# Autodesk Inventor assembly: mg996r_bottom
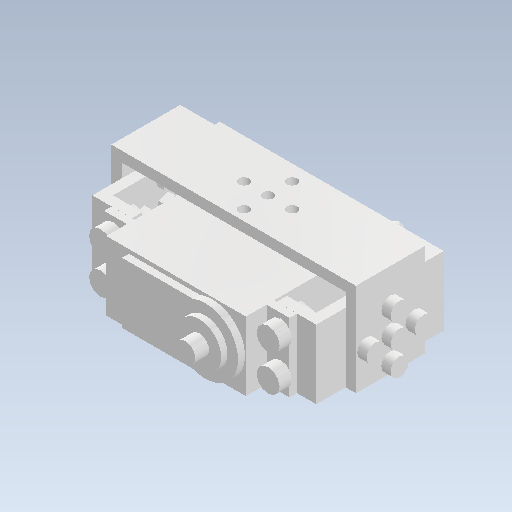
[picture p0: Inventor's stored thumbnail of the model, 512x512]
Saved by Autodesk Inventor 2021.4 (Build 254397000, 397)
## iProperties
Created: 2022-07-25
Part Number: mg996r_bottom
Document SubType Name: Assembly
Designer: isamu
Author: isamu
## Documents named in this file (5)
- D:\personal_projects\robot\inventor\2021_matlab_compat\mg996r_bottom.iam
- D:\personal_projects\robot\inventor\2021_matlab_compat\mg996r_servo_frame_with_axis.iam
- D:\personal_projects\robot\exports\frames\servo frame part 3.ipt
- D:\personal_projects\robot\exports\screws\m3x8.ipt
- D:\personal_projects\robot\exports\screws\m3 nuts.ipt
## Components (22 placed, 4 different names)
1. mg996r_servo_frame_with_axis:1 [sub-assembly] — Mate:1, Mate:2, Mate:3, Insert:11, Insert:12, Insert:13, Insert:14, Insert:15, Insert:16, Insert:17, Insert:18, Insert:19, Insert:20
2. servo frame part 3:1 — Mate:1, Mate:2, Mate:3, Insert:1, Insert:2, Insert:3, Insert:4, Insert:5, Insert:6, Insert:7, Insert:8, Insert:9, Insert:10
3. m3x8:1 — Insert:7
4. m3x8:2 — Insert:8
5. m3x8:3 — Insert:10
6. m3x8:4 — Insert:9
7. m3x8:5 — Insert:6
8. m3x8:6 — Insert:2
9. m3x8:7 — Insert:3
10. m3x8:8 — Insert:5
11. m3x8:9 — Insert:4
12. m3x8:10 — Insert:1
13. m3 nuts:1 — Insert:17
14. m3 nuts:2 — Insert:20
15. m3 nuts:3 — Insert:19
16. m3 nuts:4 — Insert:16
17. m3 nuts:5 — Insert:18
18. m3 nuts:6 — Insert:11
19. m3 nuts:7 — Insert:14
20. m3 nuts:8 — Insert:13
21. m3 nuts:9 — Insert:15
22. m3 nuts:10 — Insert:12
## Relationships (23: Insert 20, Mate 3)
- Mate:1: mg996r_servo_frame_with_axis:1 ↔ servo frame part 3:1
- Mate:2: mg996r_servo_frame_with_axis:1 ↔ servo frame part 3:1
- Mate:3: mg996r_servo_frame_with_axis:1 ↔ servo frame part 3:1
- Insert:1: servo frame part 3:1 ↔ m3x8:10
- Insert:2: servo frame part 3:1 ↔ m3x8:6
- Insert:3: servo frame part 3:1 ↔ m3x8:7
- Insert:4: servo frame part 3:1 ↔ m3x8:9
- Insert:5: servo frame part 3:1 ↔ m3x8:8
- Insert:6: servo frame part 3:1 ↔ m3x8:5
- Insert:7: servo frame part 3:1 ↔ m3x8:1
- Insert:8: servo frame part 3:1 ↔ m3x8:2
- Insert:9: servo frame part 3:1 ↔ m3x8:4
- Insert:10: servo frame part 3:1 ↔ m3x8:3
- Insert:11: mg996r_servo_frame_with_axis:1 ↔ m3 nuts:6
- Insert:12: mg996r_servo_frame_with_axis:1 ↔ m3 nuts:10
- Insert:13: mg996r_servo_frame_with_axis:1 ↔ m3 nuts:8
- Insert:14: mg996r_servo_frame_with_axis:1 ↔ m3 nuts:7
- Insert:15: mg996r_servo_frame_with_axis:1 ↔ m3 nuts:9
- Insert:16: mg996r_servo_frame_with_axis:1 ↔ m3 nuts:4
- Insert:17: mg996r_servo_frame_with_axis:1 ↔ m3 nuts:1
- Insert:18: mg996r_servo_frame_with_axis:1 ↔ m3 nuts:5
- Insert:19: mg996r_servo_frame_with_axis:1 ↔ m3 nuts:3
- Insert:20: mg996r_servo_frame_with_axis:1 ↔ m3 nuts:2
